# Autodesk Inventor assembly: LowerBody
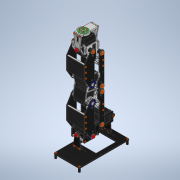
[picture p0: Inventor's stored thumbnail of the model, 180x180]
Saved by Autodesk Inventor 2020 (Build 240168000, 168)
## iProperties
Created: 2022-06-14
Part Number: LowerBody
Document SubType Name: Assembly
Designer: Masato Kubotera
Author: Masato Kubotera
## Documents named in this file (12)
- C:\Users\MasatoKubotera\Documents\Inventor\SUSTAINA-OP\LowerBody\LowerBody.iam
- C:\Users\MasatoKubotera\Documents\Inventor\SUSTAINA-OP\LowerBody\Ankle\Ankle.iam
- C:\Users\MasatoKubotera\Documents\Inventor\SUSTAINA-OP\LowerBody\Ankle\Ankle_side_pitch.iam
- C:\Users\MasatoKubotera\Documents\Inventor\SUSTAINA-OP\LowerBody\Foot\Foot.iam
- C:\Users\MasatoKubotera\Documents\Inventor\SUSTAINA-OP\LowerBody\Knee\Knee.iam
- C:\Users\MasatoKubotera\Documents\Inventor\SUSTAINA-OP\LowerBody\Leg_joint\Leg_joint_roll_pitch.iam
- C:\Users\MasatoKubotera\Documents\Inventor\SUSTAINA-OP\LowerBody\Leg_joint\Leg_joint_roll_yaw.iam
- C:\Users\MasatoKubotera\Documents\Inventor\SUSTAINA-OP\LowerBody\Link\BackLowerLink.iam
- C:\Users\MasatoKubotera\Documents\Inventor\SUSTAINA-OP\LowerBody\Link\BackUpperLink.iam
- C:\Users\MasatoKubotera\Documents\Inventor\SUSTAINA-OP\LowerBody\Link\FrontLink.iam
- C:\Users\MasatoKubotera\Documents\Inventor\SUSTAINA-OP\LowerBody\Slider_crank\Slider_crank_mechanism.iam
- C:\Users\MasatoKubotera\Documents\Inventor\SUSTAINA-OP\ReadyMade\Screw\M2_6-6.ipt
## Components (20 placed, 11 different names)
1. Leg_joint_roll_yaw:1 [sub-assembly] — フラッシュ:1, フラッシュ:2, フラッシュ:3, 挿入:1, 挿入:2, 付け根ロール軸, 付け根ロール軸:2
2. Leg_joint_roll_pitch:1 [sub-assembly] — 挿入:1, 挿入:2, 挿入:3, 挿入:4, 挿入:5, 挿入:6, 挿入:23, 付け根ロール軸
3. Slider_crank_mechanism:1 [sub-assembly] — 挿入:23, 付け根ロール軸:2
4. FrontLink:1 [sub-assembly] — 挿入:3, 挿入:4, 挿入:7, 挿入:9, 膝上ピッチ軸
5. BackUpperLink:1 [sub-assembly] — 挿入:5, 挿入:6, 挿入:8, 挿入:10
6. Knee:1 [sub-assembly] — 挿入:7, 挿入:8, 挿入:9, 挿入:10, 挿入:11, 挿入:12, 挿入:13, 挿入:14, 膝上ピッチ軸, 膝下ピッチ軸
7. BackLowerLink:1 [sub-assembly] — 挿入:13, 挿入:14, 挿入:16, 挿入:18
8. FrontLink:2 [sub-assembly] — 挿入:11, 挿入:12, 挿入:15, 挿入:17, 膝下ピッチ軸
9. Ankle:1 [sub-assembly] — 挿入:19, 挿入:20, 挿入:21, 挿入:22, 足首ピッチ軸, 足首ロール軸
10. Ankle_side_pitch:1 [sub-assembly] — 挿入:15, 挿入:16, 挿入:19, 足首ピッチ軸, 挿入:24, 挿入:25, 挿入:26, 挿入:27
11. Ankle_side_pitch:2 [sub-assembly] — 挿入:17, 挿入:18, 挿入:20, 挿入:28, 挿入:29, 挿入:30, 挿入:31
12. Foot:1 [sub-assembly] — 挿入:21, 挿入:22, 足首ロール軸
13. M2_6-6:1 — 挿入:24
14. M2_6-6:2 — 挿入:25
15. M2_6-6:3 — 挿入:26
16. M2_6-6:4 — 挿入:27
17. M2_6-6:5 — 挿入:28
18. M2_6-6:6 — 挿入:29
19. M2_6-6:7 — 挿入:30
20. M2_6-6:8 — 挿入:31
## Relationships (40: Insert 31, Angle 6, Flush 3)
- フラッシュ:1 [Flush]: Leg_joint_roll_yaw:1
- フラッシュ:2 [Flush]: Leg_joint_roll_yaw:1
- フラッシュ:3 [Flush]: Leg_joint_roll_yaw:1
- 挿入:1 [Insert]: Leg_joint_roll_yaw:1 ↔ Leg_joint_roll_pitch:1
- 挿入:2 [Insert]: Leg_joint_roll_yaw:1 ↔ Leg_joint_roll_pitch:1
- 挿入:3 [Insert]: Leg_joint_roll_pitch:1 ↔ FrontLink:1
- 挿入:4 [Insert]: Leg_joint_roll_pitch:1 ↔ FrontLink:1
- 挿入:5 [Insert]: Leg_joint_roll_pitch:1 ↔ BackUpperLink:1
- 挿入:6 [Insert]: Leg_joint_roll_pitch:1 ↔ BackUpperLink:1
- 挿入:7 [Insert]: FrontLink:1 ↔ Knee:1
- 挿入:8 [Insert]: BackUpperLink:1 ↔ Knee:1
- 挿入:9 [Insert]: FrontLink:1 ↔ Knee:1
- 挿入:10 [Insert]: BackUpperLink:1 ↔ Knee:1
- 挿入:11 [Insert]: Knee:1 ↔ FrontLink:2
- 挿入:12 [Insert]: Knee:1 ↔ FrontLink:2
- 挿入:13 [Insert]: Knee:1 ↔ BackLowerLink:1
- 挿入:14 [Insert]: Knee:1 ↔ BackLowerLink:1
- 挿入:15 [Insert]: FrontLink:2 ↔ Ankle_side_pitch:1
- 挿入:16 [Insert]: BackLowerLink:1 ↔ Ankle_side_pitch:1
- 挿入:17 [Insert]: FrontLink:2 ↔ Ankle_side_pitch:2
- 挿入:18 [Insert]: BackLowerLink:1 ↔ Ankle_side_pitch:2
- 挿入:19 [Insert]: Ankle:1 ↔ Ankle_side_pitch:1
- 挿入:20 [Insert]: Ankle:1 ↔ Ankle_side_pitch:2
- 挿入:21 [Insert]: Ankle:1 ↔ Foot:1
- 挿入:22 [Insert]: Ankle:1 ↔ Foot:1
- 挿入:23 [Insert]: Leg_joint_roll_pitch:1 ↔ Slider_crank_mechanism:1
- 付け根ロール軸 [Angle] (180 deg): Leg_joint_roll_yaw:1 ↔ Leg_joint_roll_pitch:1
- 付け根ロール軸:2 [Angle] (0 deg): Leg_joint_roll_yaw:1 ↔ Slider_crank_mechanism:1
- 膝上ピッチ軸 [Angle] (0 deg): FrontLink:1 ↔ Knee:1
- 膝下ピッチ軸 [Angle] (180 deg): Knee:1 ↔ FrontLink:2
- 足首ピッチ軸 [Angle] (0 deg): Ankle:1 ↔ Ankle_side_pitch:1
- 足首ロール軸 [Angle] (180 deg): Ankle:1 ↔ Foot:1
- 挿入:24 [Insert]: Ankle_side_pitch:1 ↔ M2_6-6:1
- 挿入:25 [Insert]: Ankle_side_pitch:1 ↔ M2_6-6:2
- 挿入:26 [Insert]: Ankle_side_pitch:1 ↔ M2_6-6:3
- 挿入:27 [Insert]: Ankle_side_pitch:1 ↔ M2_6-6:4
- 挿入:28 [Insert]: Ankle_side_pitch:2 ↔ M2_6-6:5
- 挿入:29 [Insert]: Ankle_side_pitch:2 ↔ M2_6-6:6
- 挿入:30 [Insert]: Ankle_side_pitch:2 ↔ M2_6-6:7
- 挿入:31 [Insert]: Ankle_side_pitch:2 ↔ M2_6-6:8
